# Autodesk Inventor assembly: Suporte de Talheres
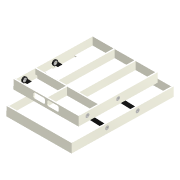
[picture p0: Inventor's stored thumbnail of the model, 180x180]
Saved by Autodesk Inventor 2020 (Build 240168000, 168)
## iProperties
Created: 2021-09-22
Part Number: Suporte de Talheres
Document SubType Name: Assembly
Designer: pablo
Author: pablo
## Documents named in this file (5)
- C:\Google Drive\Pablo Arquivos\Projetos\Utilidades Domesticas\Talheres\Suporte de Talheres.iam
- C:\Google Drive\Pablo Arquivos\Projetos\Utilidades Domesticas\Talheres\Suporte Superior.iam
- C:\Google Drive\Pablo Arquivos\Projetos\Utilidades Domesticas\Talheres\Cursor.ipt
- C:\Google Drive\Pablo Arquivos\Projetos\Utilidades Domesticas\Talheres\Suporte Inferior.iam
- C:\Google Drive\Pablo Arquivos\Projetos\Utilidades Domesticas\Talheres\Third\AIS2019\SKF_619_6-2Z.iam
## Components (14 placed, 4 different names)
1. Suporte Superior:1 [sub-assembly] — Mate:1, Mate:2, Mate:3, Mate:4, Mate:26, Mate:27
2. Cursor:1 — Mate:1, Mate:8, Mate:20, Mate:22, Mate:27
3. Cursor:2 — Mate:2, Mate:7, Mate:13, Angle:1, Mate:21, Mate:23
4. Cursor:3 — Mate:4, Mate:5, Mate:15, Mate:18, Mate:24
5. Cursor:4 — Mate:3, Mate:6, Mate:14, Mate:19, Mate:25, Mate:26
6. Suporte Inferior:1 [sub-assembly] — Mate:5, Mate:6, Mate:7, Mate:8, Mate:13, Angle:1, Mate:24, Mate:25
7. SKF_619_6-2Z:1 [sub-assembly] — Mate:14
8. SKF_619_6-2Z:2 [sub-assembly] — Mate:19
9. SKF_619_6-2Z:3 [sub-assembly] — Mate:15
10. SKF_619_6-2Z:4 [sub-assembly] — Mate:21
11. SKF_619_6-2Z:5 [sub-assembly] — Mate:22
12. SKF_619_6-2Z:6 [sub-assembly] — Mate:18
13. SKF_619_6-2Z:7 [sub-assembly] — Mate:20
14. SKF_619_6-2Z:8 [sub-assembly] — Mate:23
## Relationships (22: Mate 21, Angle 1)
- Mate:1: Suporte Superior:1 ↔ Cursor:1
- Mate:2: Suporte Superior:1 ↔ Cursor:2
- Mate:3: Suporte Superior:1 ↔ Cursor:4
- Mate:4: Suporte Superior:1 ↔ Cursor:3
- Mate:5: Cursor:3 ↔ Suporte Inferior:1
- Mate:6: Cursor:4 ↔ Suporte Inferior:1
- Mate:7: Cursor:2 ↔ Suporte Inferior:1
- Mate:8: Cursor:1 ↔ Suporte Inferior:1
- Mate:13: Cursor:2 ↔ Suporte Inferior:1
- Angle:1 (45 deg): Cursor:2 ↔ Suporte Inferior:1
- Mate:14: Cursor:4 ↔ SKF_619_6-2Z:1
- Mate:15: Cursor:3 ↔ SKF_619_6-2Z:3
- Mate:18: Cursor:3 ↔ SKF_619_6-2Z:6
- Mate:19: Cursor:4 ↔ SKF_619_6-2Z:2
- Mate:20: Cursor:1 ↔ SKF_619_6-2Z:7
- Mate:21: Cursor:2 ↔ SKF_619_6-2Z:4
- Mate:22: Cursor:1 ↔ SKF_619_6-2Z:5
- Mate:23: Cursor:2 ↔ SKF_619_6-2Z:8
- Mate:24: Cursor:3 ↔ Suporte Inferior:1
- Mate:25: Cursor:4 ↔ Suporte Inferior:1
- Mate:26: Suporte Superior:1 ↔ Cursor:4
- Mate:27: Suporte Superior:1 ↔ Cursor:1
